# Autodesk Inventor assembly: rocket_asm
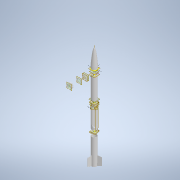
[picture p0: Inventor's stored thumbnail of the model, 180x180]
Saved by Autodesk Inventor 2020 (Build 240168000, 168)
## iProperties
Created: 2022-01-25
Part Number: rocket_asm
Document SubType Name: Assembly
Designer: sp
Author: sp
## Documents named in this file (14)
- C:\Users\sp\Documents\Rocket\rocket\CAD\rocket_asm.iam
- C:\Users\sp\Documents\Rocket\rocket\CAD\Segment_Engine.ipt
- C:\Users\sp\Documents\Rocket\rocket\CAD\Segment_mitte.ipt
- C:\Users\sp\Documents\Rocket\rocket\CAD\Segment_spitze.ipt
- C:\Users\sp\Documents\Rocket\rocket\CAD\Spitze.ipt
- C:\Users\sp\Documents\Rocket\rocket\CAD\Verbindungsring.ipt
- C:\Users\sp\Documents\Rocket\rocket\CAD\Engine.ipt
- C:\Users\sp\Documents\Rocket\rocket\CAD\Leitwerk.ipt
- C:\Users\sp\Documents\Rocket\rocket\CAD\Electro_unit.ipt
- C:\Users\sp\Documents\Rocket\rocket\CAD\Back_holder.ipt
- C:\Users\sp\Documents\Rocket\rocket\CAD\Deckel_Parachute.ipt
- C:\Users\sp\Documents\Rocket\rocket\CAD\Servo_Ku_asm.iam
- C:\Users\sp\Documents\Rocket\rocket\CAD\parachute_structure_asm.iam
- C:\Users\sp\Documents\Rocket\rocket\CAD\Elektro_asm.iam
## Components (16 placed, 13 different names)
1. Segment_Engine:1 — Passend:1, Passend:2, Passend:14
2. Segment_mitte:1 — Passend:2, Passend:3, Passend:4, Passend:5, Passend:17, Einfügen:1, Einfügen:2
3. Segment_spitze:1 — Passend:3, Passend:6
4. Spitze:1 — Passend:1
5. Verbindungsring:1 — Passend:4
6. Verbindungsring:2 — Passend:5
7. Engine:1 — Passend:6, Passend:8, Fluchtend:1, Passend:9, Passend:10, Passend:11, Fluchtend:2, Passend:12, Passend:13, Fluchtend:3, Passend:15, Passend:16
8. Leitwerk:1 — Passend:8, Fluchtend:1, Passend:9
9. Leitwerk:2 — Passend:10, Passend:11, Fluchtend:2
10. Leitwerk:3 — Passend:12, Passend:13, Fluchtend:3
11. Electro_unit:1 — Passend:14
12. Back_holder:1 — Passend:15, Passend:16
13. Deckel_Parachute:1 — Passend:17
14. Servo_Ku_asm:1 [sub-assembly] — Einfügen:1
15. parachute_structure_asm:1 [sub-assembly] — Einfügen:2
16. Elektro_asm:1 [sub-assembly]
## Relationships (21: Mate 16, Flush 3, Insert 2)
- Passend:1 [Mate]: Segment_Engine:1 ↔ Spitze:1
- Passend:2 [Mate]: Segment_Engine:1 ↔ Segment_mitte:1
- Passend:3 [Mate]: Segment_mitte:1 ↔ Segment_spitze:1
- Passend:4 [Mate]: Segment_mitte:1 ↔ Verbindungsring:1
- Passend:5 [Mate]: Segment_mitte:1 ↔ Verbindungsring:2
- Passend:6 [Mate]: Segment_spitze:1 ↔ Engine:1
- Passend:8 [Mate]: Engine:1 ↔ Leitwerk:1
- Fluchtend:1 [Flush]: Engine:1 ↔ Leitwerk:1
- Passend:9 [Mate] (10.5 mm): Engine:1 ↔ Leitwerk:1
- Passend:10 [Mate]: Engine:1 ↔ Leitwerk:2
- Passend:11 [Mate]: Engine:1 ↔ Leitwerk:2
- Fluchtend:2 [Flush]: Engine:1 ↔ Leitwerk:2
- Passend:12 [Mate]: Engine:1 ↔ Leitwerk:3
- Passend:13 [Mate]: Engine:1 ↔ Leitwerk:3
- Fluchtend:3 [Flush]: Engine:1 ↔ Leitwerk:3
- Passend:14 [Mate]: Segment_Engine:1 ↔ Electro_unit:1
- Passend:15 [Mate]: Engine:1 ↔ Back_holder:1
- Passend:16 [Mate]: Engine:1 ↔ Back_holder:1
- Passend:17 [Mate]: Segment_mitte:1 ↔ Deckel_Parachute:1
- Einfügen:1 [Insert] (20 mm): Segment_mitte:1 ↔ Servo_Ku_asm:1
- Einfügen:2 [Insert] (-250 mm): Segment_mitte:1 ↔ parachute_structure_asm:1
